# Autodesk Inventor assembly: Assembly3
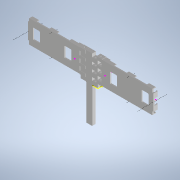
[picture p0: Inventor's stored thumbnail of the model, 180x180]
Saved by Autodesk Inventor 2020 (Build 240168000, 168)
## iProperties
Created: 2020-03-31
Part Number: Assembly3
Document SubType Name: Assembly
Designer: Sverrir
Author: Sverrir
## Documents named in this file (3)
- C:\Users\Sverrir\Desktop\Skóli\Human-Centered Artificial Intelligence\1. Semester\Computer vision\Project\3D\Assembly3.iam
- C:\Users\Sverrir\Desktop\Skóli\Human-Centered Artificial Intelligence\1. Semester\Computer vision\Project\3D\Part9 scaled.ipt
- C:\Users\Sverrir\Desktop\Skóli\Human-Centered Artificial Intelligence\1. Semester\Computer vision\Project\3D\Center.ipt
## Components (3 placed, 2 different names)
1. Part9 scaled:1 — Flush:1, Mate:1, Flush:2
2. Part9 scaled:2 — Flush:1, Flush:4, Mate:2
3. Center:1 — Mate:1, Flush:2, Flush:4, Mate:2
## Relationships (5: Flush 3, Mate 2)
- Flush:1: Part9 scaled:1 ↔ Part9 scaled:2
- Mate:1: Part9 scaled:1 ↔ Center:1
- Flush:2: Part9 scaled:1 ↔ Center:1
- Flush:4: Part9 scaled:2 ↔ Center:1
- Mate:2: Part9 scaled:2 ↔ Center:1
